# Autodesk Inventor assembly: testing_gripper
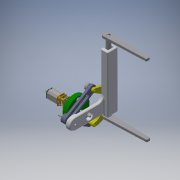
[picture p0: Inventor's stored thumbnail of the model, 180x180]
Saved by Autodesk Inventor 2017 (Build 210142000, 142)
## iProperties
Created: 2018-02-06
Part Number: testing_gripper
Document SubType Name: Assembly
Designer: Nic
Author: Nic
## Documents named in this file (16)
- C:\Users\Nic\Documents\iDripper\testing_gripper.iam
- C:\Users\Nic\Documents\iDripper\motor_shaft.ipt
- C:\Users\Nic\Documents\iDripper\slider_link_p1.ipt
- C:\Users\Nic\Documents\iDripper\slider_link_p2.ipt
- C:\Users\Nic\Documents\iDripper\slider_link_p3.ipt
- C:\Users\Nic\Documents\iDripper\slider_link_p4.ipt
- C:\Users\Nic\Documents\iDripper\slider_link_p5.ipt
- C:\Users\Nic\Documents\iDripper\slider_wheel.ipt
- C:\Users\Nic\Documents\iDripper\slider_knob_long.ipt
- C:\Users\Nic\Documents\iDripper\gripper_support.ipt
- C:\Users\Nic\Documents\iDripper\slider_link_p6.ipt
- C:\Users\Nic\Documents\HumiditySensingRig\micro-metal-gearmotor-backshaft.ipt
- C:\Users\Nic\Documents\iDripper\motor_hub.ipt
- C:\Users\Nic\Documents\iDripper\spring_knob.iam
- C:\Users\Nic\Documents\iDripper\spring_hold_p2.ipt
- C:\Users\Nic\Documents\iDripper\slider_knob.ipt
## Components (19 placed, 15 different names)
1. motor_shaft:1 — Insert:10, Insert:22
2. slider_link_p1:1 — Tangent:5, Insert:28, Insert:30
3. slider_link_p2:1 — Insert:15, Insert:27
4. slider_link_p3:1 — Tangent:3, Mate:3, Mate:8
5. slider_wheel:1 — Insert:18, Insert:19, Insert:20, Insert:21, Insert:22
6. slider_link_p1:2 — Tangent:2, Insert:27, Insert:29, Insert:30, Insert:31
7. slider_knob_long:1 — Tangent:2, Insert:20
8. slider_link_p4:1 — Insert:13, Insert:24, Insert:28
9. gripper_support:1 — Insert:10, Insert:14, Angle:1, Mate:10, Mate:11, Insert:29
10. motor_shaft:2 — Insert:14
11. slider_link_p5:1 — Insert:13, Tangent:3, Mate:3, Mate:8, Mate:11
12. slider_link_p6:1 — Insert:15, Mate:6, Tangent:4, Mate:7, Mate:10
13. slider_link_p3:2 — Mate:6, Tangent:4, Mate:7
14. slider_knob_long:2 — Tangent:5, Insert:21
15. micro-metal-gearmotor-backshaft:1 — Insert:17, Angle:1
16. motor_hub:1 — Insert:17, Insert:18, Insert:19
17. spring_knob:1 [sub-assembly] — Insert:24
18. slider_knob:1 — Insert:26, Insert:31
19. spring_hold_p2:1 — Insert:26
## Relationships (28: Insert 17, Mate 6, Tangent 4, Angle 1)
- Tangent:2: slider_link_p1:2 ↔ slider_knob_long:1
- Insert:10 (-1 mm): motor_shaft:1 ↔ gripper_support:1
- Insert:13 (3 mm): slider_link_p4:1 ↔ slider_link_p5:1
- Insert:14 (-3 mm): gripper_support:1 ↔ motor_shaft:2
- Tangent:3: slider_link_p3:1 ↔ slider_link_p5:1
- Mate:3: slider_link_p3:1 ↔ slider_link_p5:1
- Insert:15 (3 mm): slider_link_p2:1 ↔ slider_link_p6:1
- Mate:6: slider_link_p6:1 ↔ slider_link_p3:2
- Tangent:4: slider_link_p6:1 ↔ slider_link_p3:2
- Mate:7: slider_link_p6:1 ↔ slider_link_p3:2
- Tangent:5: slider_link_p1:1 ↔ slider_knob_long:2
- Mate:8: slider_link_p3:1 ↔ slider_link_p5:1
- Insert:17: micro-metal-gearmotor-backshaft:1 ↔ motor_hub:1
- Insert:18: slider_wheel:1 ↔ motor_hub:1
- Insert:19: slider_wheel:1 ↔ motor_hub:1
- Insert:20: slider_wheel:1 ↔ slider_knob_long:1
- Insert:21: slider_wheel:1 ↔ slider_knob_long:2
- Insert:22 (-2.8 mm): motor_shaft:1 ↔ slider_wheel:1
- Angle:1 (0 deg): gripper_support:1 ↔ micro-metal-gearmotor-backshaft:1
- Insert:24 (2 mm): slider_link_p4:1 ↔ spring_knob:1
- Insert:26: slider_knob:1 ↔ spring_hold_p2:1
- Insert:27: slider_link_p2:1 ↔ slider_link_p1:2
- Insert:28: slider_link_p1:1 ↔ slider_link_p4:1
- Mate:10 (2 mm): gripper_support:1 ↔ slider_link_p6:1
- Mate:11 (2 mm): gripper_support:1 ↔ slider_link_p5:1
- Insert:29 (3.5 mm): slider_link_p1:2 ↔ gripper_support:1
- Insert:30: slider_link_p1:1 ↔ slider_link_p1:2
- Insert:31: slider_link_p1:2 ↔ slider_knob:1
